# Autodesk Inventor assembly: Assy_curve_module
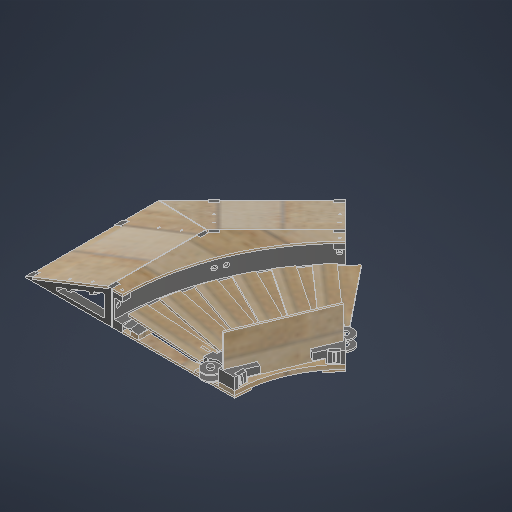
[picture p0: Inventor's stored thumbnail of the model, 512x512]
Saved by Autodesk Inventor 2026.3 (Build 303398000, 398)
## iProperties
Created: 2025-09-28
Part Number: Assy_curve_module
Document SubType Name: Assembly
Designer: hibik
Author: hibik
## Documents named in this file (15)
- D:\model\D2_Conveyor_2026\curve_module\Assy_curve_module.iam
- D:\model\D2_Conveyor_2026\curve_module\base.ipt
- D:\model\D2_Conveyor_2026\curve_module\back_under.ipt
- D:\model\D2_Conveyor_2026\curve_module\back_upper.ipt
- D:\model\D2_Conveyor_2026\curve_module\front.ipt
- D:\model\D2_Conveyor_2026\curve_module\belt_rail.ipt
- D:\model\D2_Conveyor_2026\curve_module\front_rail.ipt
- D:\model\D2_Conveyor_2026\belt\belt_curve.iam
- D:\model\D2_Conveyor_2026\connectors\connector_male_bend_left.ipt
- D:\model\D2_Conveyor_2026\connectors\connector_male_bend_right.ipt
- D:\model\D2_Conveyor_2026\curve_module\wall.ipt
- D:\model\D2_Conveyor_2026\curve_module\Right_Wall.ipt
- D:\model\D2_Conveyor_2026\curve_module\lefft_wall.ipt
- D:\model\D2_Conveyor_2026\curve_module\Spcer_curve.ipt
- D:\model\D2_Conveyor_2026\curve_module\Wall_Stand.ipt
## Components (18 placed, 14 different names)
1. base:1 — 挿入:3, 挿入:5, フラッシュ:2, 角度:8, 正接:3
2. front:1 — 挿入:3, 角度:3, フラッシュ:3, フラッシュ:4, フラッシュ:5
3. back_under:1 — 挿入:5, 角度:5, 挿入:7, フラッシュ:1, 挿入:8, 挿入:9, 正接:2, メイト:1, メイト:2, メイト:3, メイト:4, メイト:5, メイト:6, メイト:9
4. back_upper:1 — 角度:6, 挿入:9
5. base:2 — 挿入:7, フラッシュ:1
6. belt_rail:1 — 挿入:8, フラッシュ:2, 正接:1
7. front_rail:1 — フラッシュ:3, フラッシュ:4, フラッシュ:5, メイト:11, メイト:13, メイト:28, メイト:29, メイト:30, メイト:31, メイト:32, フラッシュ:6, フラッシュ:7, フラッシュ:12
8. belt_curve:1 [sub-assembly] — 正接:1, 正接:2, 角度:8, 正接:3
9. connector_male_bend_left:1 — メイト:2, メイト:3, メイト:6
10. connector_male_bend_right:1 — メイト:1, メイト:4, メイト:5, メイト:7, メイト:8
11. wall:1 — メイト:7, メイト:8, メイト:9
12. Right_Wall:1 — メイト:34, メイト:35, メイト:36, メイト:37, メイト:38, フラッシュ:8, フラッシュ:9
13. lefft_wall:1 — メイト:33, メイト:39, メイト:40, メイト:41, メイト:42, メイト:43, フラッシュ:10, フラッシュ:11
14. Spcer_curve:1 — メイト:28, フラッシュ:12
15. Wall_Stand:1 — メイト:32, メイト:34, メイト:37, フラッシュ:7, フラッシュ:9
16. Wall_Stand:2 — メイト:29, メイト:41, メイト:42, メイト:43, フラッシュ:10
17. Wall_Stand:3 — メイト:30, メイト:33, メイト:39, メイト:40, フラッシュ:6, フラッシュ:11
18. Wall_Stand:4 — メイト:31, メイト:35, メイト:36, メイト:38, フラッシュ:8
## Relationships (52: Mate 27, Flush 12, Insert 5, Angle 4, Tangent 3, Symmetry 1)
- 挿入:3 [Insert]: base:1 ↔ front:1
- 角度:3 [Angle] (0 deg): front:1
- 挿入:5 [Insert]: base:1 ↔ back_under:1
- 角度:5 [Angle] (0 deg): back_under:1
- 角度:6 [Angle] (0 deg): back_upper:1
- 挿入:7 [Insert]: back_under:1 ↔ base:2
- フラッシュ:1 [Flush]: back_under:1 ↔ base:2
- 挿入:8 [Insert]: back_under:1 ↔ belt_rail:1
- フラッシュ:2 [Flush]: base:1 ↔ belt_rail:1
- 挿入:9 [Insert]: back_under:1 ↔ back_upper:1
- フラッシュ:3 [Flush]: front:1 ↔ front_rail:1
- フラッシュ:4 [Flush]: front:1 ↔ front_rail:1
- フラッシュ:5 [Flush]: front:1 ↔ front_rail:1
- 正接:1 [Tangent]: belt_rail:1 ↔ belt_curve:1
- 正接:2 [Tangent]: back_under:1 ↔ belt_curve:1
- 角度:8 [Angle] (3.75 deg): base:1 ↔ belt_curve:1
- 正接:3 [Tangent] (-3.5 mm): base:1 ↔ belt_curve:1
- メイト:1 [Mate]: back_under:1 ↔ connector_male_bend_right:1
- メイト:2 [Mate]: back_under:1 ↔ connector_male_bend_left:1
- メイト:3 [Mate]: back_under:1 ↔ connector_male_bend_left:1
- メイト:4 [Mate]: back_under:1 ↔ connector_male_bend_right:1
- メイト:5 [Mate]: back_under:1 ↔ connector_male_bend_right:1
- メイト:6 [Mate]: back_under:1 ↔ connector_male_bend_left:1
- メイト:7 [Mate]: connector_male_bend_right:1 ↔ wall:1
- メイト:8 [Mate]: connector_male_bend_right:1 ↔ wall:1
- メイト:9 [Mate]: back_under:1 ↔ wall:1
- メイト:11 [Mate]: front_rail:1
- メイト:13 [Mate]: front_rail:1
- 対称度:1 [Symmetry]
- メイト:28 [Mate]: front_rail:1 ↔ Spcer_curve:1
- メイト:29 [Mate]: front_rail:1 ↔ Wall_Stand:2
- メイト:30 [Mate]: front_rail:1 ↔ Wall_Stand:3
- メイト:31 [Mate]: front_rail:1 ↔ Wall_Stand:4
- メイト:32 [Mate]: front_rail:1 ↔ Wall_Stand:1
- メイト:33 [Mate]: lefft_wall:1 ↔ Wall_Stand:3
- メイト:34 [Mate]: Right_Wall:1 ↔ Wall_Stand:1
- メイト:35 [Mate]: Right_Wall:1 ↔ Wall_Stand:4
- メイト:36 [Mate]: Right_Wall:1 ↔ Wall_Stand:4
- メイト:37 [Mate]: Right_Wall:1 ↔ Wall_Stand:1
- メイト:38 [Mate]: Right_Wall:1 ↔ Wall_Stand:4
- メイト:39 [Mate]: lefft_wall:1 ↔ Wall_Stand:3
- メイト:40 [Mate]: lefft_wall:1 ↔ Wall_Stand:3
- メイト:41 [Mate]: lefft_wall:1 ↔ Wall_Stand:2
- メイト:42 [Mate]: lefft_wall:1 ↔ Wall_Stand:2
- メイト:43 [Mate]: lefft_wall:1 ↔ Wall_Stand:2
- フラッシュ:6 [Flush]: front_rail:1 ↔ Wall_Stand:3
- フラッシュ:7 [Flush]: front_rail:1 ↔ Wall_Stand:1
- フラッシュ:8 [Flush]: Right_Wall:1 ↔ Wall_Stand:4
- フラッシュ:9 [Flush]: Right_Wall:1 ↔ Wall_Stand:1
- フラッシュ:10 [Flush]: lefft_wall:1 ↔ Wall_Stand:2
- フラッシュ:11 [Flush]: lefft_wall:1 ↔ Wall_Stand:3
- フラッシュ:12 [Flush]: front_rail:1 ↔ Spcer_curve:1
